# Autodesk Inventor assembly: sparAssembly
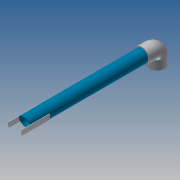
[picture p0: Inventor's stored thumbnail of the model, 180x180]
Saved by Autodesk Inventor 2014 (Build 180170000, 170)
## iProperties
Created: 2013-12-03
Part Number: sparAssembly
Document SubType Name: Assembly
Designer: Dave
Author: Dave
## Documents named in this file (4)
- C:\Users\ddeboer\Desktop\hera-cad\support\sparAssembly.iam
- C:\Users\ddeboer\Desktop\hera-cad\support\sparVert.ipt
- C:\Users\ddeboer\Desktop\hera-cad\surface\joinerBracket.ipt
- C:\Users\ddeboer\Desktop\hera-cad\smallParts\elbow_90deg_63mm.ipt
## Components (4 placed, 3 different names)
1. sparVert:1 — Insert:1, Insert:2, Insert:3
2. elbow_90deg_63mm:1 — Insert:1
3. joinerBracket:1 — Insert:2, Insert:3
4. joinerBracket:2
## Component patterns: (2 elements, first: joinerBracket:1)
## Relationships (3: Insert 3)
- Insert:1 (-38 mm): sparVert:1 ↔ elbow_90deg_63mm:1
- Insert:2: sparVert:1 ↔ joinerBracket:1
- Insert:3: sparVert:1 ↔ joinerBracket:1
